# Autodesk Inventor assembly: MagToolChanger_Tool
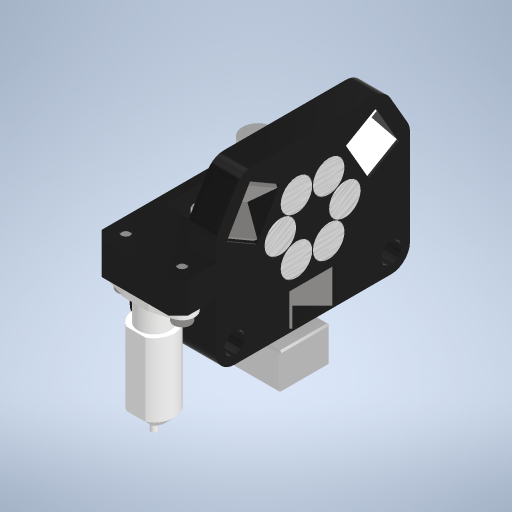
[picture p0: Inventor's stored thumbnail of the model, 512x512]
Saved by Autodesk Inventor 2023.2 (Build 272271000, 271)
## iProperties
Created: 2022-06-19
Part Number: MagToolChanger_Tool
Document SubType Name: Assembly
Designer: Remo
Author: Remo
## Documents named in this file (8)
- C:\Users\remop\OneDrive\Documents\Inventor\3D Printers\LuEVO\Mk4_Toolchanger\MagToolChanger_Tool.iam
- C:\Users\remop\OneDrive\Documents\Inventor\3D Printers\LuEVO\Mk4_Toolchanger\MagToolChanger_Tool.ipt
- C:\Users\remop\OneDrive\Documents\Inventor\3D Printers\LuEVO\Mk4_Toolchanger\MagToolChanger_CouplerL.ipt
- C:\Users\remop\OneDrive\Documents\Inventor\3D Printers\LuEVO\Mk4_Toolchanger\MagToolChanger_Magnet.ipt
- C:\Users\remop\OneDrive\Documents\Inventor\3D Printers\LuEVO\Mk4_Toolchanger\Arethusa.ipt
- C:\Users\remop\OneDrive\Documents\Inventor\Content Center Files\R2023\en-US\AS 1420\AS 1420 - 1973 - M3 x 8.ipt
- C:\Users\remop\OneDrive\Documents\Inventor\3D Printers\LuEVO\Mk4_Toolchanger\BLTouch.ipt
- C:\Users\remop\OneDrive\Documents\Inventor\Content Center Files\R2023\en-US\AS 1420\AS 1420 - 1973 - M3 x 12.ipt
## Components (18 placed, 7 different names)
1. MagToolChanger_Tool:1 — Mate:1, Mate:2, Mate:3, Mate:4, Mate:5, Mate:6, Mate:7, Mate:8, Mate:9, Rigid:1, Rigid:2, Rigid:3, Rigid:4, Rigid:5, Rigid:6, Mate:10, Flush:1, Mate:11, Insert:1, Insert:2, Insert:3, Insert:4, Rigid:8
2. MagToolChanger_CouplerL:1 — Mate:4, Mate:5, Mate:6
3. MagToolChanger_CouplerL:3 — Mate:7, Mate:8, Mate:9
4. MagToolChanger_CouplerL:2 — Mate:1, Mate:2, Mate:3
5. MagToolChanger_Magnet:1 — Rigid:1
6. MagToolChanger_Magnet:2 — Rigid:2
7. MagToolChanger_Magnet:3 — Rigid:3
8. MagToolChanger_Magnet:4 — Rigid:4
9. MagToolChanger_Magnet:5 — Rigid:5
10. MagToolChanger_Magnet:6 — Rigid:6
11. Arethusa:1 — Mate:10, Flush:1, Mate:11
12. AS 1420 - Metric M3 x 8:1 — Insert:1
13. AS 1420 - Metric M3 x 8:2 — Insert:2
14. AS 1420 - Metric M3 x 8:3 — Insert:3
15. AS 1420 - Metric M3 x 8:4 — Insert:4
16. BLTouch:1 — Rigid:8, Insert:5, Insert:6
17. AS 1420 - Metric M3 x 12:1 — Insert:5
18. AS 1420 - Metric M3 x 12:2 — Insert:6
## Relationships (25: Mate 11, WeldJoint 7, Insert 6, Flush 1)
- Mate:1: MagToolChanger_Tool:1 ↔ MagToolChanger_CouplerL:2
- Mate:2: MagToolChanger_Tool:1 ↔ MagToolChanger_CouplerL:2
- Mate:3: MagToolChanger_Tool:1 ↔ MagToolChanger_CouplerL:2
- Mate:4: MagToolChanger_Tool:1 ↔ MagToolChanger_CouplerL:1
- Mate:5: MagToolChanger_Tool:1 ↔ MagToolChanger_CouplerL:1
- Mate:6: MagToolChanger_Tool:1 ↔ MagToolChanger_CouplerL:1
- Mate:7: MagToolChanger_Tool:1 ↔ MagToolChanger_CouplerL:3
- Mate:8: MagToolChanger_Tool:1 ↔ MagToolChanger_CouplerL:3
- Mate:9: MagToolChanger_Tool:1 ↔ MagToolChanger_CouplerL:3
- Rigid:1 [WeldJoint]: MagToolChanger_Tool:1 ↔ MagToolChanger_Magnet:1
- Rigid:2 [WeldJoint]: MagToolChanger_Tool:1 ↔ MagToolChanger_Magnet:2
- Rigid:3 [WeldJoint]: MagToolChanger_Tool:1 ↔ MagToolChanger_Magnet:3
- Rigid:4 [WeldJoint]: MagToolChanger_Tool:1 ↔ MagToolChanger_Magnet:4
- Rigid:5 [WeldJoint]: MagToolChanger_Tool:1 ↔ MagToolChanger_Magnet:5
- Rigid:6 [WeldJoint]: MagToolChanger_Tool:1 ↔ MagToolChanger_Magnet:6
- Mate:10: MagToolChanger_Tool:1 ↔ Arethusa:1
- Flush:1 (-3 mm): MagToolChanger_Tool:1 ↔ Arethusa:1
- Mate:11 (8 mm): MagToolChanger_Tool:1 ↔ Arethusa:1
- Insert:1: MagToolChanger_Tool:1 ↔ AS 1420 - Metric M3 x 8:1
- Insert:2: MagToolChanger_Tool:1 ↔ AS 1420 - Metric M3 x 8:2
- Insert:3: MagToolChanger_Tool:1 ↔ AS 1420 - Metric M3 x 8:3
- Insert:4: MagToolChanger_Tool:1 ↔ AS 1420 - Metric M3 x 8:4
- Rigid:8 [WeldJoint]: MagToolChanger_Tool:1 ↔ BLTouch:1
- Insert:5: BLTouch:1 ↔ AS 1420 - Metric M3 x 12:1
- Insert:6: BLTouch:1 ↔ AS 1420 - Metric M3 x 12:2
